# Autodesk Inventor assembly: testframe
(part 2 of 2)
- Mate:394: STRU_018_AngleBracket_62:1 ↔ COTS_90044A124_Black-Oxide Alloy Steel Socket Head Screw:5
- Mate:395: STRU_018_AngleBracket_62:1 ↔ COTS_90044A124_Black-Oxide Alloy Steel Socket Head Screw:6
- Mate:396: STRU_018_AngleBracket_62:1 ↔ COTS_90044A124_Black-Oxide Alloy Steel Socket Head Screw:10
- Mate:397: STRU_018_AngleBracket_62:1 ↔ COTS_90044A124_Black-Oxide Alloy Steel Socket Head Screw:11
- Mate:398: STRU_018_AngleBracket_62:1 ↔ COTS_90044A124_Black-Oxide Alloy Steel Socket Head Screw:12
- Mate:399: STRU_018_AngleBracket_62:1 ↔ COTS_90044A124_Black-Oxide Alloy Steel Socket Head Screw:4
- Mate:400: STRU_018_AngleBracket_62:1 ↔ COTS_90044A124_Black-Oxide Alloy Steel Socket Head Screw:6
- Mate:401: STRU_018_AngleBracket_62:1 ↔ COTS_90044A124_Black-Oxide Alloy Steel Socket Head Screw:5
- Mate:402: STRU_018_AngleBracket_62:1 ↔ COTS_90044A124_Black-Oxide Alloy Steel Socket Head Screw:12
- Mate:403: STRU_018_AngleBracket_62:1 ↔ COTS_90044A124_Black-Oxide Alloy Steel Socket Head Screw:11
- Mate:404: STRU_018_AngleBracket_62:1 ↔ COTS_90044A124_Black-Oxide Alloy Steel Socket Head Screw:10
- Mate:408: STRU_003_BilletPole_28in_Angled_Unique:1 ↔ STRU_010_BilletCrossbar_Angled:2
- Mate:409: STRU_011_BilletWedge:4 ↔ STRU_010_BilletCrossbar_Angled:2
- Mate:410: STRU_011_BilletWedge:5 ↔ STRU_010_BilletCrossbar_Angled:2
- Mate:411: STRU_002_BilletPole_20.56in_Angled:1 ↔ STRU_010_BilletCrossbar_Angled:2
- Mate:412: STRU_003_BilletPole_28in_Angled_Unique:1 ↔ STRU_010_BilletCrossbar_Angled:3
- Mate:413: STRU_011_BilletWedge:3 ↔ STRU_010_BilletCrossbar_Angled:3
- Mate:414: STRU_011_BilletWedge:1 ↔ STRU_010_BilletCrossbar_Angled:3
- Mate:415: STRU_002_BilletPole_20.56in_Angled:2 ↔ STRU_010_BilletCrossbar_Angled:3
- Mate:416: STRU_012_BilletPoleMiddle:5 ↔ COTS_90044A123_Black-Oxide Alloy Steel Socket Head Screw:30
- Mate:417: STRU_012_BilletPoleMiddle:5 ↔ COTS_90044A123_Black-Oxide Alloy Steel Socket Head Screw:29
- Mate:418: STRU_012_BilletPoleMiddle:6 ↔ COTS_90044A123_Black-Oxide Alloy Steel Socket Head Screw:28
- Mate:419: STRU_012_BilletPoleMiddle:6 ↔ COTS_90044A123_Black-Oxide Alloy Steel Socket Head Screw:27
- Mate:420: COTS_90044A124_Black-Oxide Alloy Steel Socket Head Screw:12 ↔ COTS_95615A120_Medium-Strength Steel Nylon-Insert Locknut:34
- Mate:421: COTS_90044A124_Black-Oxide Alloy Steel Socket Head Screw:4 ↔ COTS_95615A120_Medium-Strength Steel Nylon-Insert Locknut:32
- Mate:422: COTS_90044A124_Black-Oxide Alloy Steel Socket Head Screw:5 ↔ COTS_95615A120_Medium-Strength Steel Nylon-Insert Locknut:35
- Mate:423: COTS_90044A124_Black-Oxide Alloy Steel Socket Head Screw:6 ↔ COTS_95615A120_Medium-Strength Steel Nylon-Insert Locknut:31
- Mate:424: COTS_90044A124_Black-Oxide Alloy Steel Socket Head Screw:11 ↔ COTS_95615A120_Medium-Strength Steel Nylon-Insert Locknut:36
- Mate:425: COTS_90044A124_Black-Oxide Alloy Steel Socket Head Screw:10 ↔ COTS_95615A120_Medium-Strength Steel Nylon-Insert Locknut:33
- Mate:426: STRU_018_AngleBracket_62:3 ↔ COTS_95615A120_Medium-Strength Steel Nylon-Insert Locknut:32
- Mate:427: STRU_018_AngleBracket_62:3 ↔ COTS_95615A120_Medium-Strength Steel Nylon-Insert Locknut:34
- Mate:428: STRU_018_AngleBracket_62:3 ↔ COTS_95615A120_Medium-Strength Steel Nylon-Insert Locknut:36
- Mate:429: STRU_018_AngleBracket_62:3 ↔ COTS_95615A120_Medium-Strength Steel Nylon-Insert Locknut:33
- Mate:430: STRU_018_AngleBracket_62:3 ↔ COTS_95615A120_Medium-Strength Steel Nylon-Insert Locknut:31
- Mate:431: STRU_018_AngleBracket_62:3 ↔ COTS_95615A120_Medium-Strength Steel Nylon-Insert Locknut:35
- Mate:432: COTS_91251A539_Black-Oxide Alloy Steel Socket Head Screw (1):2 ↔ COTS_95462A029_Medium-Strength Steel Hex Nut (2):1
- Mate:433: COTS_91251A539_Black-Oxide Alloy Steel Socket Head Screw (1):2 ↔ STRU_019_RubberWasher:1
- Mate:434: STRU_017_AngleBracket_90_Plastic:2 ↔ STRU_019_RubberWasher:1
- Mate:435: STRU_017_AngleBracket_90_Plastic:2 ↔ STRU_019_RubberWasher:1
- Mate:436: COTS_95462A029_Medium-Strength Steel Hex Nut (2):1 ↔ STRU_019_RubberWasher:1
- [Mate]: COTS_95462A029_Medium-Strength Steel Hex Nut (2):2 ↔ STRU_019_RubberWasher:2
- Mate:438: COTS_95462A029_Medium-Strength Steel Hex Nut (2):2 ↔ STRU_019_RubberWasher:2
- Mate:439: COTS_91251A539_Black-Oxide Alloy Steel Socket Head Screw (1):1 ↔ COTS_95462A029_Medium-Strength Steel Hex Nut (2):2
- Flush:59: STRU_019_RubberWasher:1 ↔ STRU_019_RubberWasher:2
- Mate:440: STRU_017_AngleBracket_90_Plastic:2 ↔ STRU_019_RubberWasher:2
- [Mate]: COTS_95462A029_Medium-Strength Steel Hex Nut (2):3 ↔ STRU_019_RubberWasher:3
- Mate:442: COTS_90044A123_Black-Oxide Alloy Steel Socket Head Screw:30 ↔ COTS_95462A029_Medium-Strength Steel Hex Nut (2):3
- Mate:443: COTS_90044A123_Black-Oxide Alloy Steel Socket Head Screw:30 ↔ STRU_019_RubberWasher:3
- Mate:444: STRU_017_AngleBracket_90_Plastic:2 ↔ STRU_019_RubberWasher:3
- Mate:445: STRU_017_AngleBracket_90_Plastic:2 ↔ STRU_019_RubberWasher:3
- [Mate]: COTS_95462A029_Medium-Strength Steel Hex Nut (2):4 ↔ STRU_019_RubberWasher:4
- Mate:447: COTS_95462A029_Medium-Strength Steel Hex Nut (2):4 ↔ STRU_019_RubberWasher:4
- Mate:448: COTS_90044A123_Black-Oxide Alloy Steel Socket Head Screw:29 ↔ COTS_95462A029_Medium-Strength Steel Hex Nut (2):4
- Mate:449: STRU_017_AngleBracket_90_Plastic:2 ↔ STRU_019_RubberWasher:4
- Flush:60: STRU_019_RubberWasher:3 ↔ STRU_019_RubberWasher:4
- [Mate]: COTS_95462A029_Medium-Strength Steel Hex Nut (2):5 ↔ STRU_019_RubberWasher:5
- [Mate]: COTS_95462A029_Medium-Strength Steel Hex Nut (2):5 ↔ STRU_019_RubberWasher:5
- Mate:452: COTS_91251A539_Black-Oxide Alloy Steel Socket Head Screw (1):5 ↔ COTS_95462A029_Medium-Strength Steel Hex Nut (2):5
- Mate:453: STRU_017_AngleBracket_90_Plastic:1 ↔ STRU_019_RubberWasher:5
- Mate:454: STRU_017_AngleBracket_90_Plastic:1 ↔ STRU_019_RubberWasher:5
- [Mate]: COTS_95462A029_Medium-Strength Steel Hex Nut (2):6 ↔ STRU_019_RubberWasher:6
- [Mate]: COTS_95462A029_Medium-Strength Steel Hex Nut (2):6 ↔ STRU_019_RubberWasher:6
- Mate:457: COTS_91251A539_Black-Oxide Alloy Steel Socket Head Screw (1):4 ↔ COTS_95462A029_Medium-Strength Steel Hex Nut (2):6
- Mate:458: STRU_017_AngleBracket_90_Plastic:1 ↔ STRU_019_RubberWasher:6
- Flush:61: STRU_019_RubberWasher:5 ↔ STRU_019_RubberWasher:6
- [Mate]: COTS_95462A029_Medium-Strength Steel Hex Nut (2):7 ↔ STRU_019_RubberWasher:7
- [Mate]: COTS_95462A029_Medium-Strength Steel Hex Nut (2):7 ↔ STRU_019_RubberWasher:7
- Mate:461: COTS_90044A123_Black-Oxide Alloy Steel Socket Head Screw:27 ↔ COTS_95462A029_Medium-Strength Steel Hex Nut (2):7
- Mate:462: STRU_017_AngleBracket_90_Plastic:1 ↔ STRU_019_RubberWasher:7
- Mate:463: STRU_017_AngleBracket_90_Plastic:1 ↔ STRU_019_RubberWasher:7
- [Mate]: COTS_95462A029_Medium-Strength Steel Hex Nut (2):8 ↔ STRU_019_RubberWasher:8
- [Mate]: COTS_95462A029_Medium-Strength Steel Hex Nut (2):8 ↔ STRU_019_RubberWasher:8
- Mate:466: COTS_90044A123_Black-Oxide Alloy Steel Socket Head Screw:28 ↔ COTS_95462A029_Medium-Strength Steel Hex Nut (2):8
- Mate:467: STRU_017_AngleBracket_90_Plastic:1 ↔ STRU_019_RubberWasher:8
- Flush:62: STRU_019_RubberWasher:7 ↔ STRU_019_RubberWasher:8
## Named parameters: d22_d7 = 0 mm, d23_d8 = 0 mm, d24_d9 = 0 mm, d25_d10 = 0 mm, d26_d11 = 0 mm, d27_d12 = 0 mm, d389_d130 = 0 mm, d393_d130 = 0 mm, d397_d130 = 0 mm, d401_d130 = 0 mm, d405_d130 = 0 mm, d409_d130 = 0 mm, d413_d130 = 0 mm, d417_d130 = 0 mm, sa_0 = 981, sa_1 = 11120.6, sa_2 = 11120.6, sa_3 = 11120.6, sa_4 = 11120.6, d560_d559 = 0 mm, d565_d559 = 0 mm, d570_d559 = 0 mm, d575_d570_d559 = 0 mm, d576_d571 = 0 mm, d580_d575_d570_d559 = 0 mm, d581_d576_d571 = 0 mm, d585_d575_d570_d559 = 0 mm, d586_d576_d571 = 0 mm, d590_d575_d570_d559 = 0 mm, d591_d576_d571 = 0 mm
note: some values were not read from the file. Shown as the stored number, unit unknown: "sa_0", "sa_1", "sa_2", "sa_3", "sa_4".
